# Autodesk Inventor assembly: Spindle_Block_ASM_MIR
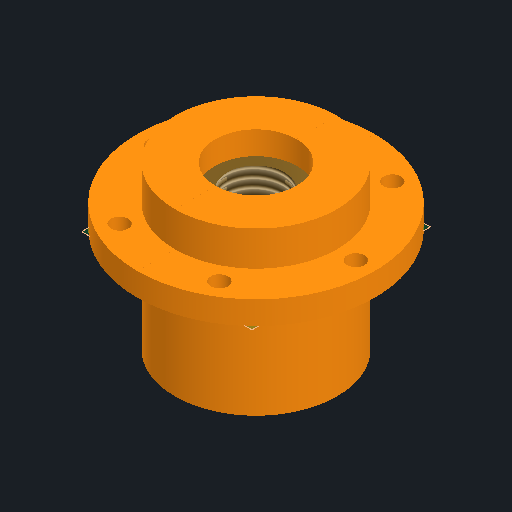
[picture p0: Inventor's stored thumbnail of the model, 512x512]
Saved by Autodesk Inventor 2024.1 (Build 281209000, 209)
## iProperties
Created: 2023-08-04
Part Number: Spindle_Block_ASM_MIR
Document SubType Name: Assembly
Designer: jaege
Author: jaege
## Documents named in this file (3)
- C:\Users\jaege\VUB\Schakel_Ind_Elo\Year_1_Both\BA_Thesis\3D_Files\Lift_V2\Spindle_Block_ASM_MIR.iam
- C:\Users\jaege\VUB\Schakel_Ind_Elo\Year_1_Both\BA_Thesis\3D_Files\Lift_V2\SpindleBlock_MIR.ipt
- C:\Users\jaege\VUB\Schakel_Ind_Elo\Year_1_Both\BA_Thesis\3D_Files\Lift_V2\Spindle_Block_Holder_MIR.ipt
## Components (3 placed, 2 different names)
1. SpindleBlock_MIR:1 — Mate:1, Mate:2, Mate:5, Mate:4
2. Spindle_Block_Holder_MIR:1 — Mate:1, Mate:2, Mate:3
3. Spindle_Block_Holder_MIR:2 — Mate:5, Mate:3, Mate:4
## Relationships (5: Mate 5)
- Mate:1: SpindleBlock_MIR:1 ↔ Spindle_Block_Holder_MIR:1
- Mate:2: SpindleBlock_MIR:1 ↔ Spindle_Block_Holder_MIR:1
- Mate:5: SpindleBlock_MIR:1 ↔ Spindle_Block_Holder_MIR:2
- Mate:3: Spindle_Block_Holder_MIR:1 ↔ Spindle_Block_Holder_MIR:2
- Mate:4: SpindleBlock_MIR:1 ↔ Spindle_Block_Holder_MIR:2
